# Autodesk Inventor assembly: Assembly1
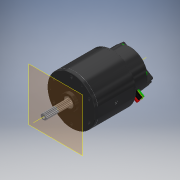
[picture p0: Inventor's stored thumbnail of the model, 180x180]
Saved by Autodesk Inventor 2019 (Build 230136000, 136)
## iProperties
Created: 2020-01-08
Part Number: Assembly1
Document SubType Name: Assembly
Designer: mavericks
Author: mavericks
## Documents named in this file (2)
- T:\EIT\2020 Infinite Recharge\2020 ROBOT\COMMON PARTS\SPACERS\Assembly1.iam
- T:\EIT\2020 Infinite Recharge\2020 ROBOT\COMMON PARTS\MOTORS\Falcon_500_Powered_by_Talon_FX_217-6515 (1).ipt
## Components (1 placed, 1 different names)
1. Falcon_500_Powered_by_Talon_FX_217-6515 (1):1 — Mate:1, Angle:1
## Relationships (2: Mate 1, Angle 1)
- Mate:1: Falcon_500_Powered_by_Talon_FX_217-6515 (1):1
- Angle:1 (0 deg): Falcon_500_Powered_by_Talon_FX_217-6515 (1):1
